# Autodesk Inventor assembly: Rig_v1
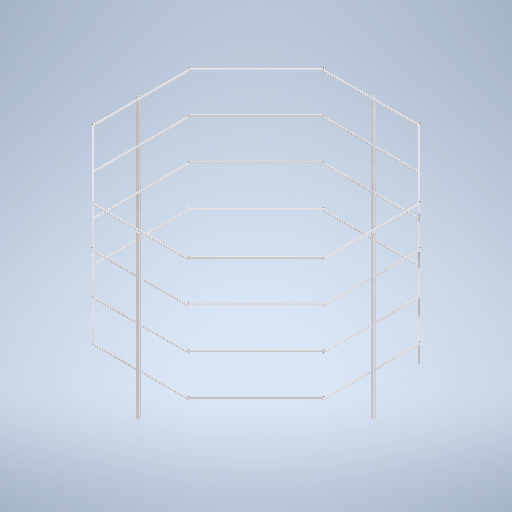
[picture p0: Inventor's stored thumbnail of the model, 512x512]
Saved by Autodesk Inventor 2025.1 (Build 291241000, 241)
## iProperties
Created: 2024-10-13
Part Number: Rig_v1
Document SubType Name: Assembly
Designer: Kai Altwicker
Author: Kai Altwicker
## Documents named in this file (8)
- C:\Users\tallA\Repos\VolumanXR\hardware-capture\cad\rig_v1\Rig_v1.iam
- C:\Users\tallA\Repos\VolumanXR\hardware-capture\cad\rig_v1\Segment_Staender_v1.iam
- C:\Users\tallA\Repos\VolumanXR\hardware-capture\cad\rig_v1\Segment_Traeger_v1.iam
- Z:\WINDOWS\Documents\Inventor\Content Center Files\R2025\de-DE\DIN 603\DIN 603 - M5 x 50.ipt
- Z:\WINDOWS\Documents\Inventor\Content Center Files\R2025\de-DE\DIN 9021\DIN 9021 - 5,3.ipt
- Z:\WINDOWS\Documents\Inventor\Content Center Files\R2025\de-DE\DIN 1587\DIN 1587 - M5 x 0,8.ipt
- C:\Users\tallA\Repos\VolumanXR\hardware-capture\cad\rig_v1\Segment_Traeger_Tuer_v1.iam
- C:\Users\tallA\Repos\VolumanXR\hardware-capture\cad\dimensions.xlsx
## Components (200 placed, 6 different names)
1. Segment_Traeger_Tuer_v1:1 [sub-assembly] — Passend:8, Passend:9, Passend:10
2. Segment_Staender_v1:1 [sub-assembly] — Fluchtend:1, Passend:1, Fluchtend:2, Passend:2, Winkel:1, Passend:3, Passend:8
3. Segment_Staender_v1:2 [sub-assembly]
4. Segment_Staender_v1:3 [sub-assembly]
5. Segment_Staender_v1:4 [sub-assembly] — Passend:4, Passend:5, Passend:9, Passend:10
6. Segment_Traeger_v1:1 [sub-assembly] — Passend:2, Winkel:1, Passend:3
7. Segment_Traeger_v1:2 [sub-assembly]
8. Segment_Traeger_v1:3 [sub-assembly] — Passend:7
9. DIN 603 M5 x 50:1 — Passend:4, Passend:5, Passend:6
10. DIN 9021 5,3:1 — Passend:6, Passend:7, Einfügen:1
11. DIN 1587 M5:1 — Einfügen:1
12. DIN 603 M5 x 50:2
13. DIN 9021 5,3:2
14. DIN 1587 M5:2
15. DIN 603 M5 x 50:3
16. DIN 9021 5,3:3
17. DIN 1587 M5:3
18. DIN 603 M5 x 50:4
19. DIN 9021 5,3:4
20. DIN 1587 M5:4
21. DIN 603 M5 x 50:5
22. DIN 9021 5,3:5
23. DIN 1587 M5:5
24. DIN 603 M5 x 50:6
25. DIN 9021 5,3:6
26. DIN 1587 M5:6
27. DIN 603 M5 x 50:7
28. DIN 9021 5,3:7
29. DIN 1587 M5:7
30. DIN 603 M5 x 50:8
31. DIN 9021 5,3:8
32. DIN 1587 M5:8
33. DIN 603 M5 x 50:9
34. DIN 9021 5,3:9
35. DIN 1587 M5:9
36. DIN 603 M5 x 50:10
37. DIN 9021 5,3:10
38. DIN 1587 M5:10
39. DIN 603 M5 x 50:11
40. DIN 9021 5,3:11
41. DIN 1587 M5:11
42. DIN 603 M5 x 50:12
43. DIN 9021 5,3:12
44. DIN 1587 M5:12
45. DIN 603 M5 x 50:13
46. DIN 9021 5,3:13
47. DIN 1587 M5:13
48. DIN 603 M5 x 50:14
49. DIN 9021 5,3:14
50. DIN 1587 M5:14
51. DIN 603 M5 x 50:15
52. DIN 9021 5,3:15
53. DIN 1587 M5:15
54. DIN 603 M5 x 50:16
55. DIN 9021 5,3:16
56. DIN 1587 M5:16
57. DIN 603 M5 x 50:17
58. DIN 9021 5,3:17
59. DIN 1587 M5:17
60. DIN 603 M5 x 50:18
61. DIN 9021 5,3:18
62. DIN 1587 M5:18
63. DIN 603 M5 x 50:19
64. DIN 9021 5,3:19
65. DIN 1587 M5:19
66. DIN 603 M5 x 50:20
67. DIN 9021 5,3:20
68. DIN 1587 M5:20
69. DIN 603 M5 x 50:21
70. DIN 9021 5,3:21
71. DIN 1587 M5:21
72. DIN 603 M5 x 50:22
73. DIN 9021 5,3:22
74. DIN 1587 M5:22
75. DIN 603 M5 x 50:23
76. DIN 9021 5,3:23
77. DIN 1587 M5:23
78. DIN 603 M5 x 50:24
79. DIN 9021 5,3:24
80. DIN 1587 M5:24
81. DIN 603 M5 x 50:25
82. DIN 9021 5,3:25
83. DIN 1587 M5:25
84. DIN 603 M5 x 50:26
85. DIN 9021 5,3:26
86. DIN 1587 M5:26
87. DIN 603 M5 x 50:27
88. DIN 9021 5,3:27
89. DIN 1587 M5:27
90. DIN 603 M5 x 50:28
91. DIN 9021 5,3:28
92. DIN 1587 M5:28
93. DIN 603 M5 x 50:29
94. DIN 9021 5,3:29
95. DIN 1587 M5:29
96. DIN 603 M5 x 50:30
97. DIN 9021 5,3:30
98. DIN 1587 M5:30
99. DIN 603 M5 x 50:31
100. DIN 9021 5,3:31
101. DIN 1587 M5:31
102. DIN 603 M5 x 50:32
103. DIN 9021 5,3:32
104. DIN 1587 M5:32
105. DIN 603 M5 x 50:33
106. DIN 9021 5,3:33
107. DIN 1587 M5:33
108. DIN 603 M5 x 50:34
109. DIN 9021 5,3:34
110. DIN 1587 M5:34
111. DIN 603 M5 x 50:35
112. DIN 9021 5,3:35
113. DIN 1587 M5:35
114. DIN 603 M5 x 50:36
115. DIN 9021 5,3:36
116. DIN 1587 M5:36
117. DIN 603 M5 x 50:37
118. DIN 9021 5,3:37
119. DIN 1587 M5:37
120. DIN 603 M5 x 50:38
121. DIN 9021 5,3:38
122. DIN 1587 M5:38
123. DIN 603 M5 x 50:39
124. DIN 9021 5,3:39
125. DIN 1587 M5:39
126. DIN 603 M5 x 50:40
127. DIN 9021 5,3:40
128. DIN 1587 M5:40
129. DIN 603 M5 x 50:41
130. DIN 9021 5,3:41
131. DIN 1587 M5:41
132. DIN 603 M5 x 50:42
133. DIN 9021 5,3:42
134. DIN 1587 M5:42
135. DIN 603 M5 x 50:43
136. DIN 9021 5,3:43
137. DIN 1587 M5:43
138. DIN 603 M5 x 50:44
139. DIN 9021 5,3:44
140. DIN 1587 M5:44
141. DIN 603 M5 x 50:45
142. DIN 9021 5,3:45
143. DIN 1587 M5:45
144. DIN 603 M5 x 50:46
145. DIN 9021 5,3:46
146. DIN 1587 M5:46
147. DIN 603 M5 x 50:47
148. DIN 9021 5,3:47
149. DIN 1587 M5:47
150. DIN 603 M5 x 50:48
151. DIN 9021 5,3:48
152. DIN 1587 M5:48
153. DIN 603 M5 x 50:49
154. DIN 9021 5,3:49
155. DIN 1587 M5:49
156. DIN 603 M5 x 50:50
157. DIN 9021 5,3:50
158. DIN 1587 M5:50
159. DIN 603 M5 x 50:51
160. DIN 9021 5,3:51
161. DIN 1587 M5:51
162. DIN 603 M5 x 50:52
163. DIN 9021 5,3:52
164. DIN 1587 M5:52
165. DIN 603 M5 x 50:53
166. DIN 9021 5,3:53
167. DIN 1587 M5:53
168. DIN 603 M5 x 50:54
169. DIN 9021 5,3:54
170. DIN 1587 M5:54
171. DIN 603 M5 x 50:55
172. DIN 9021 5,3:55
173. DIN 1587 M5:55
174. DIN 603 M5 x 50:56
175. DIN 9021 5,3:56
176. DIN 1587 M5:56
177. DIN 603 M5 x 50:57
178. DIN 9021 5,3:57
179. DIN 1587 M5:57
180. DIN 603 M5 x 50:58
181. DIN 9021 5,3:58
182. DIN 1587 M5:58
183. DIN 603 M5 x 50:59
184. DIN 9021 5,3:59
185. DIN 1587 M5:59
186. DIN 603 M5 x 50:60
187. DIN 9021 5,3:60
188. DIN 1587 M5:60
189. DIN 603 M5 x 50:61
190. DIN 9021 5,3:61
191. DIN 1587 M5:61
192. DIN 603 M5 x 50:62
193. DIN 9021 5,3:62
194. DIN 1587 M5:62
195. DIN 603 M5 x 50:63
196. DIN 9021 5,3:63
197. DIN 1587 M5:63
198. DIN 603 M5 x 50:64
199. DIN 9021 5,3:64
200. DIN 1587 M5:64
## Component patterns: (4 elements, first: Segment_Staender_v1:1), (3 elements, first: Segment_Traeger_v1:1), (16 elements), (4 elements, first: DIN 603 M5 x 50:1 + DIN 9021 5,3:1 + DIN 1587 M5:1), Komponentenanordnung 5:2 (4 elements), Komponentenanordnung 5:3 (4 elements), Komponentenanordnung 5:4 (4 elements), Komponentenanordnung 5:5 (4 elements), Komponentenanordnung 5:6 (4 elements), Komponentenanordnung 5:7 (4 elements), Komponentenanordnung 5:8 (4 elements), Komponentenanordnung 5:9 (4 elements), Komponentenanordnung 5:10 (4 elements), Komponentenanordnung 5:11 (4 elements), Komponentenanordnung 5:12 (4 elements), Komponentenanordnung 5:13 (4 elements), Komponentenanordnung 5:14 (4 elements), Komponentenanordnung 5:15 (4 elements), Komponentenanordnung 5:16 (4 elements)
## Relationships (14: Mate 10, Flush 2, Angle 1, Insert 1)
- Fluchtend:1 [Flush] (1796.518 mm): Segment_Staender_v1:1
- Passend:1 [Mate]: Segment_Staender_v1:1
- Fluchtend:2 [Flush]: Segment_Staender_v1:1
- Passend:2 [Mate]: Segment_Staender_v1:1 ↔ Segment_Traeger_v1:1
- Winkel:1 [Angle] (-45 deg): Segment_Staender_v1:1 ↔ Segment_Traeger_v1:1
- Passend:3 [Mate]: Segment_Staender_v1:1 ↔ Segment_Traeger_v1:1
- Passend:4 [Mate]: Segment_Staender_v1:4 ↔ DIN 603 M5 x 50:1
- Passend:5 [Mate]: Segment_Staender_v1:4 ↔ DIN 603 M5 x 50:1
- Passend:6 [Mate]: DIN 603 M5 x 50:1 ↔ DIN 9021 5,3:1
- Passend:7 [Mate]: Segment_Traeger_v1:3 ↔ DIN 9021 5,3:1
- Einfügen:1 [Insert]: DIN 9021 5,3:1 ↔ DIN 1587 M5:1
- Passend:8 [Mate]: Segment_Traeger_Tuer_v1:1 ↔ Segment_Staender_v1:1
- Passend:9 [Mate]: Segment_Traeger_Tuer_v1:1 ↔ Segment_Staender_v1:4
- Passend:10 [Mate]: Segment_Traeger_Tuer_v1:1 ↔ Segment_Staender_v1:4
## Named parameters: d_tol = 0.3 mm, d_wand = 1.5 mm, l_profil_40x40 = 2500 mm, h_profil_40x40 = 40 mm, h_profil_20x20 = 20 mm, d_traeger = 625 mm, b_profil_40x40 = 40 mm, b_profil_20x20 = 20 mm, l_profil_20x20 = 1500 mm, D_oct = 3573.03607 mm
